# Autodesk Inventor assembly: FieldFinal
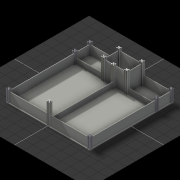
[picture p0: Inventor's stored thumbnail of the model, 180x180]
Saved by Autodesk Inventor 2016 (Build 200138000, 138)
## iProperties
Created: 2017-01-21
Part Number: FieldFinal
Document SubType Name: Assembly
Designer: Alexis Renderos
Author: Alexis Renderos
## Documents named in this file (15)
- C:\Users\Alexis Renderos\Documents\Lego Robotics Missions\FieldFinal.iam
- C:\Users\Alexis Renderos\Documents\Lego Robotics Missions\PolyBase.ipt
- C:\Users\Alexis Renderos\Documents\Lego Robotics Missions\ProfileOne.ipt
- C:\Users\Alexis Renderos\Documents\Lego Robotics Missions\NLNMNMNR.ipt
- C:\Users\Alexis Renderos\Documents\Lego Robotics Missions\NLMFLNRMFR.ipt
- C:\Users\Alexis Renderos\Documents\Lego Robotics Missions\NLMFLNRMFR_MIR.ipt
- C:\Users\Alexis Renderos\Documents\Lego Robotics Missions\MFLSLMFRSR.ipt
- C:\Users\Alexis Renderos\Documents\Lego Robotics Missions\MFLSLMFRSR_MIR.ipt
- C:\Users\Alexis Renderos\Documents\Lego Robotics Missions\SLSMLSMRSR.ipt
- C:\Users\Alexis Renderos\Documents\Lego Robotics Missions\SLSMLSMRSR_MIR.ipt
- C:\Users\Alexis Renderos\Documents\Lego Robotics Missions\MLSMLMRSMR.ipt
- C:\Users\Alexis Renderos\Documents\Lego Robotics Missions\MFLMLMRMFR.ipt
- C:\Users\Alexis Renderos\Documents\Lego Robotics Missions\MLMRSMLSMR.ipt
- C:\Users\Alexis Renderos\Documents\Lego Robotics Missions\ProfileTwo.ipt
- C:\Users\Alexis Renderos\Documents\Lego Robotics Missions\DividerDown.ipt
## Components (28 placed, 27 different names)
1. PolyBase:1 — Mate:5, Mate:6, Mate:7, Mate:8, Mate:9, Mate:10, Flush:9, Flush:10, Flush:14, Mate:19, Mate:20, Mate:21, Mate:24, Mate:27, Mate:29, Mate:33, Mate:35, Mate:37, Mate:39, Mate:48, Mate:50, Mate:53, Mate:56, Mate:59, Mate:60, Mate:61, Mate:62
2. NorthLeft
3. NorthMiddle — Mate:10, Flush:14, Mate:23, Mate:26
4. NorthRight
5. MiddleFarLeft — Mate:60
6. MiddleLeft — Mate:9, Flush:11, Flush:13, Symmetry:1, Mate:17
7. MiddleCenter — Mate:8, Flush:13, Flush:15, Mate:63, Flush:27
8. MiddleRight — Mate:7, Flush:12, Symmetry:1, Flush:15, Mate:54, Mate:55
9. MiddleFarRight — Mate:61
10. SouthLeft
11. SouthMiddleLeft — Mate:5, Flush:9, Flush:11, Mate:17, Mate:19, Mate:49, Flush:24
12. SouthMiddleRight — Mate:6, Flush:10, Flush:12, Mate:51, Mate:52, Mate:57, Mate:58, Mate:59
13. SouthRight
14. NL-NM — Mate:20, Mate:23
15. NM-NR — Mate:21, Mate:24, Mate:26
16. NL-MFL — Mate:27
17. NR-MFR — Mate:39
18. MFL-SL — Mate:29
19. MFR-SR — Mate:37
20. SL-SML — Mate:33
21. SMR-SR — Mate:35
22. MFL-ML
23. MR-MFR
24. ML-SML — Mate:48, Mate:49, Flush:24
25. MR-SMR — Mate:50, Mate:51, Mate:52
26. MLMRSMLSMR:1 — Mate:53, Mate:54, Mate:55
27. MLMRSMLSMR:2 — Mate:56, Mate:57, Mate:58
28. DividerDown:1 — Mate:62, Mate:63, Flush:27
## Relationships (87: Mate 58, Flush 27, Symmetry 2)
- [Mate]: PolyBase:1 ↔ SouthRight
- [Flush]: PolyBase:1 ↔ SouthRight
- [Flush]: PolyBase:1 ↔ SouthRight
- [Mate]: PolyBase:1 ↔ SouthLeft
- [Flush]: PolyBase:1 ↔ SouthLeft
- [Flush]: PolyBase:1 ↔ SouthLeft
- [Mate]: PolyBase:1 ↔ NorthRight
- [Flush]: PolyBase:1 ↔ NorthRight
- [Flush]: PolyBase:1 ↔ NorthRight
- [Mate]: PolyBase:1 ↔ NorthLeft
- [Flush]: PolyBase:1 ↔ NorthLeft
- [Flush]: PolyBase:1 ↔ NorthLeft
- Mate:5: PolyBase:1 ↔ SouthMiddleLeft
- Mate:6: PolyBase:1 ↔ SouthMiddleRight
- Mate:7: PolyBase:1 ↔ MiddleRight
- Mate:8: PolyBase:1 ↔ MiddleCenter
- Mate:9: PolyBase:1 ↔ MiddleLeft
- Mate:10: PolyBase:1 ↔ NorthMiddle
- Flush:9: PolyBase:1 ↔ SouthMiddleLeft
- Flush:10: PolyBase:1 ↔ SouthMiddleRight
- Flush:11: MiddleLeft ↔ SouthMiddleLeft
- Flush:12: MiddleRight ↔ SouthMiddleRight
- Flush:13: MiddleLeft ↔ MiddleCenter
- Symmetry:1: MiddleLeft ↔ MiddleRight
- Flush:14: PolyBase:1 ↔ NorthMiddle
- [Symmetry]: NorthLeft ↔ NorthRight
- Flush:15: MiddleCenter ↔ MiddleRight
- [Mate] (304.8 mm): SouthLeft ↔ SouthMiddleLeft
- [Mate] (304.8 mm): SouthMiddleRight ↔ SouthRight
- [Mate]: PolyBase:1 ↔ MiddleFarLeft
- [Flush]: PolyBase:1 ↔ MiddleFarLeft
- [Flush]: MiddleFarLeft ↔ MiddleLeft
- [Mate]: PolyBase:1 ↔ MiddleFarRight
- [Flush]: PolyBase:1 ↔ MiddleFarRight
- [Flush]: MiddleRight ↔ MiddleFarRight
- Mate:17 (152.4 mm): MiddleLeft ↔ SouthMiddleLeft
- [Mate]: PolyBase:1 ↔ MiddleFarLeft
- Mate:19: PolyBase:1 ↔ SouthMiddleLeft
- Mate:20: PolyBase:1 ↔ NL-NM
- Mate:21: PolyBase:1 ↔ NM-NR
- [Mate]: NorthLeft ↔ NL-NM
- Mate:23: NorthMiddle ↔ NL-NM
- Mate:24: PolyBase:1 ↔ NM-NR
- [Mate]: NorthRight ↔ NM-NR
- Mate:26: NorthMiddle ↔ NM-NR
- Mate:27: PolyBase:1 ↔ NL-MFL
- [Mate]: NorthLeft ↔ NL-MFL
- [Flush]: NorthLeft ↔ NL-MFL
- Mate:29: PolyBase:1 ↔ MFL-SL
- [Mate]: SouthLeft ↔ MFL-SL
- [Mate]: SouthLeft ↔ MFL-SL
- Mate:33: PolyBase:1 ↔ SL-SML
- [Mate]: SouthLeft ↔ SL-SML
- [Flush]: SouthLeft ↔ SL-SML
- Mate:35: PolyBase:1 ↔ SMR-SR
- [Mate]: SouthRight ↔ SMR-SR
- [Flush]: SouthRight ↔ SMR-SR
- Mate:37: PolyBase:1 ↔ MFR-SR
- [Mate]: SouthRight ↔ MFR-SR
- [Flush]: SouthRight ↔ MFR-SR
- Mate:39: PolyBase:1 ↔ NR-MFR
- [Mate]: NorthRight ↔ NR-MFR
- [Mate]: NorthRight ↔ NR-MFR
- [Mate]: PolyBase:1 ↔ MFL-ML
- [Mate]: MiddleFarLeft ↔ MFL-ML
- [Mate]: PolyBase:1 ↔ MR-MFR
- [Mate]: MiddleFarRight ↔ MR-MFR
- Mate:48: PolyBase:1 ↔ ML-SML
- Mate:49: SouthMiddleLeft ↔ ML-SML
- Flush:24: SouthMiddleLeft ↔ ML-SML
- [Flush]: MiddleFarLeft ↔ MFL-ML
- [Flush]: MiddleFarRight ↔ MR-MFR
- Mate:50: PolyBase:1 ↔ MR-SMR
- Mate:51: SouthMiddleRight ↔ MR-SMR
- Mate:52: SouthMiddleRight ↔ MR-SMR
- Mate:53: PolyBase:1 ↔ MLMRSMLSMR:1
- Mate:54: MiddleRight ↔ MLMRSMLSMR:1
- Mate:55: MiddleRight ↔ MLMRSMLSMR:1
- Mate:56: PolyBase:1 ↔ MLMRSMLSMR:2
- Mate:57: SouthMiddleRight ↔ MLMRSMLSMR:2
- Mate:58: SouthMiddleRight ↔ MLMRSMLSMR:2
- Mate:59: PolyBase:1 ↔ SouthMiddleRight
- Mate:60: PolyBase:1 ↔ MiddleFarLeft
- Mate:61: PolyBase:1 ↔ MiddleFarRight
- Mate:62: PolyBase:1 ↔ DividerDown:1
- Mate:63: MiddleCenter ↔ DividerDown:1
- Flush:27: MiddleCenter ↔ DividerDown:1
